# Autodesk Inventor assembly: wheel_hub_mirrored
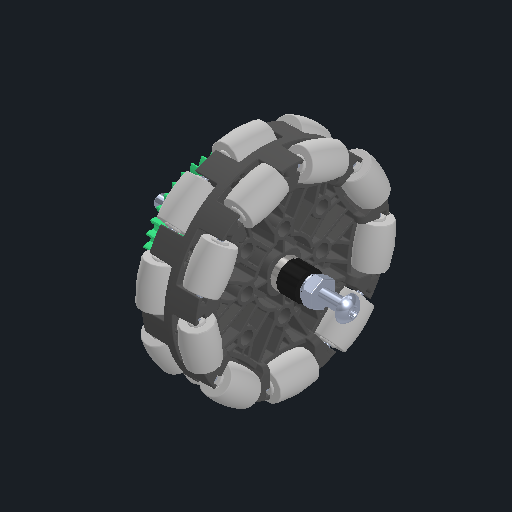
[picture p0: Inventor's stored thumbnail of the model, 512x512]
Saved by Autodesk Inventor 2025 (Build 290162000, 162)
## iProperties
Created: 2024-08-21
Part Number: wheel_hub_mirrored
Document SubType Name: Assembly
Designer: averey
Author: averey
## Documents named in this file (11)
- D:\vex_robotics_high_stakes\hardware\cad\bots\ENIGMA\chassis\drivetrain\drivebay_mirrored\wheel_hub_mirrored.iam
- D:\vex_robotics_high_stakes\hardware\cad\bots\ENIGMA\chassis\drivetrain\drivebay_mirrored\2.75 Omni AS, No Insert_mirrored.iam
- D:\vex_robotics_high_stakes\hardware\cad\VEX-CAD-Inventor\Motion\Spacers\Spacer Nylon .375 OD\NSpacer .375 OD x .250.ipt
- C:\Users\avere\vex_robotics_high_stakes\hardware\cad\VEX-CAD-Inventor\Motion\Spacers\Spacer Nylon .375 OD.ipt
- D:\vex_robotics_high_stakes\hardware\cad\VEX-CAD-Inventor\Motion\Spacers\Washer Steel\SWasher .375 OD x .062500.ipt
- C:\Users\avere\vex_robotics_high_stakes\hardware\cad\VEX-CAD-Inventor\Motion\Spacers\Washer Steel.ipt
- D:\vex_robotics_high_stakes\hardware\cad\VEX-CAD-Inventor\Motion\Spacers\Washer Steel\SWasher .375 OD x .015625.ipt
- D:\vex_robotics_high_stakes\hardware\cad\bots\ENIGMA\chassis\drivetrain\drivebay_mirrored\Nut Thin Nylock_mirrored.ipt
- D:\vex_robotics_high_stakes\hardware\cad\VEX-CAD-Inventor\Structure\Hardware\Screw Steel - Star\SScrew Star Smooth 2.500.ipt
- C:\Users\avere\vex_robotics_high_stakes\hardware\cad\VEX-CAD-Inventor\Structure\Hardware\Screw Steel - Star.ipt
- D:\vex_robotics_high_stakes\hardware\cad\bots\ENIGMA\chassis\drivetrain\drivebay_mirrored\LS 36T Gear_mirrored.ipt
## Components (7 placed, 7 different names)
1. 2.75 Omni AS, No Insert_mirrored:1 [sub-assembly] — Insert:3, Insert:6
2. NSpacer .375 OD x .250:1 — Insert:1, Insert:4
3. SWasher .375 OD x .062500:1 — Insert:1, Insert:2
4. SWasher .375 OD x .015625:2 — Insert:3, Insert:2
5. Nut Thin Nylock_mirrored:1 — Insert:4, Insert:5
6. SScrew Star Smooth 2.500:1 — Insert:5
7. LS 36T Gear_mirrored:1 — Insert:6
## Relationships (6: Insert 6)
- Insert:1: NSpacer .375 OD x .250:1 ↔ SWasher .375 OD x .062500:1
- Insert:3: 2.75 Omni AS, No Insert_mirrored:1 ↔ SWasher .375 OD x .015625:2
- Insert:2: SWasher .375 OD x .062500:1 ↔ SWasher .375 OD x .015625:2
- Insert:4: NSpacer .375 OD x .250:1 ↔ Nut Thin Nylock_mirrored:1
- Insert:5 (7.9375 mm): Nut Thin Nylock_mirrored:1 ↔ SScrew Star Smooth 2.500:1
- Insert:6 (7.1437 mm): 2.75 Omni AS, No Insert_mirrored:1 ↔ LS 36T Gear_mirrored:1
